# Autodesk Inventor assembly: SerenityMk2Complete
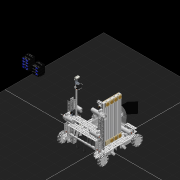
[picture p0: Inventor's stored thumbnail of the model, 180x180]
Saved by Autodesk Inventor 2015 SP1 (Build 190203100, 203)
## iProperties
Created: 2015-01-22
Part Number: SerenityMk2Complete
Document SubType Name: Assembly
Designer: rihoobler
Author: rihoobler
## Documents named in this file (41)
- C:\Users\datenney\Documents\GitHub\CAD\SerenityMk.2\SerenityMk2Complete.iam
- C:\Users\datenney\Documents\GitHub\CAD\SerenityMk.2\Frame.iam
- C:\Users\datenney\Documents\GitHub\CAD\SerenityMk.2\Normal Wheel Assembly.iam
- C:\Users\datenney\Documents\GitHub\CAD\SerenityMk.2\Omni Assembly.iam
- C:\Users\datenney\Documents\GitHub\CAD\SerenityMk.2\Imported Components\tetrix_739172_2012\tetrix_739172_2012.iam
- C:\Users\datenney\Documents\GitHub\CAD\SerenityMk.2\20X40long.ipt
- C:\Users\datenney\Documents\GitHub\CAD\SerenityMk.2\Slider.ipt
- C:\Users\datenney\Documents\GitHub\CAD\SerenityMk.2\Imported Components\tetrix_739067_2012_160_channel\tetrix_739067_2012_160_channel.ipt
- C:\Users\datenney\Documents\GitHub\CAD\SerenityMk.2\SlideAssembly.iam
- C:\Users\datenney\Documents\GitHub\CAD\SerenityMk.2\20x20extrusion.ipt
- C:\Users\datenney\Documents\GitHub\CAD\SerenityMk.2\spool.ipt
- C:\Users\datenney\Documents\GitHub\CAD\SerenityMk.2\20x20extrusionshort.ipt
- C:\Users\datenney\Documents\GitHub\CAD\SerenityMk.2\Imported Components\tetrix_739062_2012\tetrix_739062_2012.ipt
- C:\Users\datenney\Documents\GitHub\CAD\SerenityMk.2\Bucket.ipt
- C:\Users\datenney\Documents\GitHub\CAD\SerenityMk.2\Bucket Flap.ipt
- C:\Users\datenney\Documents\GitHub\CAD\SerenityMk.2\Imported Components\tetrix_739060_2012\tetrix_739060_2012.ipt
- C:\Users\datenney\Documents\GitHub\CAD\SerenityMk.2\Imported Components\tetrix_739197_2012\tetrix_739197_2012.iam
- C:\Users\datenney\Documents\GitHub\CAD\SerenityMk.2\Flat-7.ipt
- C:\Users\datenney\Documents\GitHub\CAD\SerenityMk.2\Imported Components\tetrix_739066_2012_96_channel\tetrix_739066_2012_96_channel.ipt
- C:\Users\datenney\Documents\GitHub\CAD\SerenityMk.2\ramp.ipt
- C:\Users\datenney\Documents\GitHub\CAD\SerenityMk.2\Imported Components\tetrix_739069_2012_416_channel\tetrix_739069_2012_416_channel.ipt
- C:\Users\datenney\Documents\GitHub\CAD\SerenityMk.2\Imported Components\tetrix_739068_2012_288_channel\tetrix_739068_2012_288_channel.ipt
- C:\Users\datenney\Documents\GitHub\CAD\SerenityMk.2\Imported Components\tetrix_739091_2012\tetrix_739091_2012.ipt
- C:\Users\datenney\Documents\GitHub\CAD\SerenityMk.2\sweeper.iam
- C:\Users\datenney\Documents\GitHub\CAD\SerenityMk.2\Imported Components\tetrix_739070_2012\tetrix_739070_2012.ipt
- C:\Users\datenney\Documents\GitHub\CAD\SerenityMk.2\Imported Components\sensor_light_2012\sensor_light_2012.ipt
- C:\Users\datenney\Documents\GitHub\CAD\SerenityMk.2\Imported Components\tetrix_739072_2012\tetrix_739072_2012.ipt
- C:\Users\datenney\Documents\GitHub\CAD\SerenityMk.2\Imported Components\tetrix_739089_2012\tetrix_739089_2012.ipt
- C:\Users\datenney\Documents\GitHub\CAD\SerenityMk.2\LiftSpool.ipt
- C:\Users\datenney\Documents\GitHub\CAD\COTSParts\Tetrix\Tetrix DC motor controller.ipt
- C:\Users\datenney\Documents\GitHub\CAD\COTSParts\Tetrix\NXT brick.ipt
- C:\Users\datenney\Documents\GitHub\CAD\COTSParts\Tetrix\NXT battery cover.ipt
- C:\Users\datenney\Documents\GitHub\CAD\COTSParts\Tetrix\Tetrix servo controller.ipt
- C:\Users\datenney\Documents\GitHub\CAD\COTSParts\Tetrix\Tetrix power switch.ipt
- C:\Users\datenney\Documents\GitHub\CAD\SerenityMk.2\Tetrix flat bar 257.175 mm.ipt
- C:\Users\datenney\Documents\GitHub\CAD\SerenityMk.2\Imported Components\tetrix_739197_2012\TETRIX_739197_SERVO_2012.ipt
- C:\Users\datenney\Documents\GitHub\CAD\SerenityMk.2\Imported Components\tetrix_739197_2012\TETRIX_739197_METAL_HORN_2012.ipt
- C:\Users\datenney\Documents\GitHub\CAD\SerenityMk.2\Imported Components\tetrix_739197_2012\TETRIX_739197_SCREW_2012.ipt
- C:\Users\datenney\Documents\GitHub\CAD\SerenityMk.2\Imported Components\tetrix_739197_2012\TETRIX_739197_PLASTIC_HORN_2012.ipt
- C:\Users\datenney\Documents\GitHub\CAD\SerenityMk.2\The Law Head.ipt
- C:\Users\datenney\Documents\GitHub\CAD\Imported Components\am-2964NeveRest\am-2964NeveRest.ipt
## Components (99 placed, 40 different names)
1. Frame:1 [sub-assembly] — Insert:1, Insert:2, Insert:3, Insert:4, Insert:5, Insert:6, Insert:7, Insert:8, Insert:9, Insert:10, Insert:11, Insert:12, Insert:13, Insert:14, Insert:15, Insert:16, Mate:1, Mate:2, Flush:1, Mate:6, Flush:5, Mate:7, Mate:33, Mate:34, Mate:35, Mate:42, Mate:43, Angle:8, Mate:44, Mate:45, Flush:26, Flush:27, Mate:55, Flush:29, Mate:75, Mate:76, Angle:15, Mate:84, Mate:85, Mate:86, Mate:94, Mate:95, Angle:18, Mate:111
2. Normal Wheel Assembly:1 [sub-assembly] — Insert:1
3. Normal Wheel Assembly:2 [sub-assembly] — Insert:2
4. Normal Wheel Assembly:3 [sub-assembly] — Insert:4
5. Normal Wheel Assembly:4 [sub-assembly] — Insert:3
6. Omni Assembly:1 [sub-assembly] — Insert:6, Mate:107
7. Omni Assembly:2 [sub-assembly] — Insert:5, Mate:108
8. Omni Assembly:3 [sub-assembly] — Insert:8, Mate:107, Rotation:1
9. Omni Assembly:4 [sub-assembly] — Insert:7, Mate:108, Rotation:1
10. tetrix_739172_2012:1 [sub-assembly] — Insert:9
11. tetrix_739172_2012:2 [sub-assembly] — Insert:10
12. tetrix_739172_2012:3 [sub-assembly] — Insert:11
13. tetrix_739172_2012:4 [sub-assembly] — Insert:12
14. tetrix_739172_2012:5 [sub-assembly] — Insert:15
15. tetrix_739172_2012:6 [sub-assembly] — Insert:16
16. tetrix_739172_2012:7 [sub-assembly] — Insert:13
17. tetrix_739172_2012:8 [sub-assembly] — Insert:14
18. 20X40long:1 — Mate:1, Mate:2, Flush:1, Flush:2, Mate:3, Mate:4, Mate:5, Mate:8, Mate:96, Mate:97, Flush:38
19. Slider:1 — Flush:2, Mate:3, Mate:4, Flush:4, Angle:1, Mate:9, Flush:7, Insert:17, Flush:44
20. Slider:2 — Flush:4, Mate:5, Flush:44
21. tetrix_739067_2012_160_channel:1 — Mate:6, Flush:5, Mate:7, Mate:74, Flush:28
22. SlideAssembly:1 [sub-assembly] — Angle:1, Mate:8, Mate:9, Flush:7, Angle:2, Mate:10, Flush:8, Mate:11, Insert:18
23. SlideAssembly:2 [sub-assembly] — Angle:2, Mate:10, Flush:8, Mate:11, Angle:3, Flush:9, Flush:10, Mate:12, Insert:19, Insert:20
24. SlideAssembly:3 [sub-assembly] — Angle:3, Flush:9, Flush:10, Mate:12, Angle:4, Flush:14, Flush:15, Mate:17, Insert:21, Insert:22
25. 20x20extrusion:1 — Mate:13, Mate:14, Flush:11, Mate:15, Mate:16, Flush:16, Mate:18, Flush:18
26. Slider:3 — Mate:13, Mate:14, Flush:11, Flush:12, Flush:13, Flush:14, Flush:15, Mate:17, Insert:23
27. Slider:4 — Flush:12, Flush:13, Mate:15, Mate:16, Angle:4
28. spool:1 — Insert:18
29. spool:2 — Insert:17
30. spool:3 — Insert:19
31. spool:4 — Insert:20
32. spool:6 — Insert:21
33. spool:7 — Insert:22
34. spool:8 — Insert:23
35. 20x20extrusionshort:1 — Flush:16, Mate:18, Mate:19, Angle:5, Flush:17, Flush:18, Flush:19, Mate:24, Angle:6, Flush:21
36. tetrix_739062_2012:1 — Mate:19, Angle:5, Flush:17, Mate:20, Mate:21, Mate:22
37. Bucket:1 — Mate:20, Mate:21, Mate:22, Flush:19, Flush:20, Mate:23
38. Bucket Flap:1 — Flush:20, Mate:23, Mate:31, Mate:32
39. tetrix_739060_2012:1 — Mate:24, Angle:6, Flush:21, Mate:25, Angle:7, Mate:26
40. tetrix_739197_2012:1 [sub-assembly] — Mate:25, Angle:7, Mate:26, Mate:27, Mate:28
41. Flat-7:1 — Mate:27, Mate:28, Mate:29, Mate:30
42. Flat-7:2 — Mate:29, Mate:30, Mate:31, Mate:32
43. tetrix_739066_2012_96_channel:1 — Mate:33, Mate:34, Mate:35, Mate:36, Mate:37, Mate:38
44. tetrix_739066_2012_96_channel:2 — Mate:36, Mate:37, Mate:38, Mate:39, Flush:39, Flush:40
45. ramp:1 — Mate:39, Flush:39, Flush:40
46. tetrix_739069_2012_416_channel:1 — Mate:42, Mate:43, Angle:8, Flush:22, Angle:9, Mate:46, Mate:48, Flush:24, Mate:49, Mate:56
47. tetrix_739068_2012_288_channel:1 — Flush:22, Angle:9, Mate:44, Mate:45, Mate:47, Flush:23, Mate:50, Mate:51, Flush:25, Mate:57
48. tetrix_739068_2012_288_channel:2 — Mate:46, Mate:47, Flush:23, Mate:58, Mate:59, Mate:60
49. tetrix_739068_2012_288_channel:3 — Mate:48, Flush:24, Mate:49, Mate:52, Mate:53, Mate:87, Mate:88, Mate:89, Mate:90, Mate:91, Angle:17, Mate:110, Flush:43
50. tetrix_739068_2012_288_channel:4 — Mate:50, Mate:51, Flush:25, Mate:54, Mate:92, Mate:93
51. tetrix_739066_2012_96_channel:3 — Mate:52, Mate:53, Flush:26, Angle:10, Insert:26, Insert:27
52. tetrix_739066_2012_96_channel:4 — Mate:54, Flush:27, Mate:55, Insert:24, Insert:25
53. tetrix_739068_2012_288_channel:5 — Mate:56, Angle:10, Mate:57
54. tetrix_739091_2012:1 — Insert:24
55. tetrix_739091_2012:2 — Insert:25
56. tetrix_739091_2012:3 — Insert:26, Insert:28
57. tetrix_739091_2012:4 — Insert:27
58. sweeper:1 [sub-assembly] — Insert:28
59. tetrix_739060_2012:2 — Mate:58, Mate:59, Mate:60, Mate:61, Angle:11, Mate:62
60. tetrix_739197_2012:2 [sub-assembly] — Mate:61, Angle:11, Mate:62, Mate:63, Mate:124, Mate:125
61. tetrix_739070_2012:1 — Mate:63, Mate:65, Mate:66, Mate:67, Mate:124, Mate:125
62. tetrix_739060_2012:3 — Mate:65, Mate:66, Mate:67, Mate:131, Flush:45, Mate:132
63. tetrix_739197_2012:3 [sub-assembly] — Mate:71, Mate:126, Mate:127, Mate:128, Mate:131, Flush:45, Mate:132
64. tetrix_739062_2012:2 — Mate:71, Mate:72, Mate:73, Angle:14, Mate:126, Mate:127, Mate:128
65. sensor_light_2012:1 — Mate:72, Mate:73, Angle:14
66. 20x20extrusion:2 — Mate:74, Flush:28, Flush:29
67. tetrix_739060_2012:4 — Mate:75, Mate:76, Angle:15, Mate:77, Angle:16, Mate:78
68. tetrix_739197_2012:4 [sub-assembly] — Mate:77, Angle:16, Mate:78, Mate:79, Mate:80, Mate:136, Mate:137
69. tetrix_739062_2012:3 — Mate:79, Mate:80, Mate:82, Mate:105, Mate:106, Mate:136, Mate:137
70. tetrix_739072_2012:1 — Mate:82, Mate:105, Mate:106
71. tetrix_739089_2012:1 — Mate:90, Mate:91, Angle:17, Flush:31, Mate:148, Mate:149
72. tetrix_739089_2012:2 — Flush:30, Mate:92, Mate:93, Mate:138, Mate:139
73. tetrix_739089_2012:3 — Mate:87, Mate:88, Mate:89, Flush:30, Mate:146, Mate:150
74. tetrix_739089_2012:4 — Mate:84, Mate:85, Mate:86, Mate:144, Mate:145
75. tetrix_739089_2012:5 — Mate:94, Mate:95, Angle:18, Mate:142, Mate:143
76. tetrix_739089_2012:6 — Mate:96, Mate:97, Flush:31, Mate:140, Mate:141
77. am-2964NeveRest:1 — Mate:138, Mate:139
78. am-2964NeveRest:2 — Mate:142, Mate:143
79. am-2964NeveRest:3 — Mate:146, Mate:150
80. am-2964NeveRest:4 — Mate:140, Mate:141
81. am-2964NeveRest:5 — Mate:144, Mate:145
82. am-2964NeveRest:6 — Mate:148, Mate:149
83. LiftSpool:1 — Flush:38
84. Tetrix DC motor controller:1
85. Tetrix DC motor controller:2
86. Tetrix DC motor controller:3
87. Tetrix DC motor controller:4
88. NXT brick:1 — Mate:109, Flush:41, Flush:42, Flush:43, Mate:111
89. NXT battery cover:1 — Mate:109, Flush:41, Flush:42, Mate:110
90. Tetrix servo controller:1
91. Tetrix servo controller:2
92. Tetrix servo controller:3
93. Tetrix power switch:1
94. Tetrix flat bar 257.175 mm:1 — Mate:121, Mate:122, Mate:123, Mate:133, Mate:134, Mate:135
95. TETRIX_739197_SERVO_2012:1 — Insert:29, Mate:118, Mate:120
96. TETRIX_739197_METAL_HORN_2012:1 — Mate:115, Mate:116, Mate:117, Mate:119, Mate:121, Mate:122, Mate:123, Rotation:2
97. TETRIX_739197_SCREW_2012:1 — Mate:117, Insert:29, Mate:118, Mate:119
98. TETRIX_739197_PLASTIC_HORN_2012:1 — Mate:115, Mate:116, Mate:120, Rotation:2
99. The Law Head:1 — Mate:133, Mate:134, Mate:135
## Relationships (213: Mate 129, Flush 37, Insert 29, Angle 16, RelateRotation 2)
- Insert:1: Frame:1 ↔ Normal Wheel Assembly:1
- Insert:2: Frame:1 ↔ Normal Wheel Assembly:2
- Insert:3: Frame:1 ↔ Normal Wheel Assembly:4
- Insert:4: Frame:1 ↔ Normal Wheel Assembly:3
- Insert:5: Frame:1 ↔ Omni Assembly:2
- Insert:6: Frame:1 ↔ Omni Assembly:1
- Insert:7: Frame:1 ↔ Omni Assembly:4
- Insert:8: Frame:1 ↔ Omni Assembly:3
- Insert:9: Frame:1 ↔ tetrix_739172_2012:1
- Insert:10: Frame:1 ↔ tetrix_739172_2012:2
- Insert:11: Frame:1 ↔ tetrix_739172_2012:3
- Insert:12: Frame:1 ↔ tetrix_739172_2012:4
- Insert:13: Frame:1 ↔ tetrix_739172_2012:7
- Insert:14: Frame:1 ↔ tetrix_739172_2012:8
- Insert:15: Frame:1 ↔ tetrix_739172_2012:5
- Insert:16: Frame:1 ↔ tetrix_739172_2012:6
- Mate:1: Frame:1 ↔ 20X40long:1
- Mate:2 (38.608 mm): Frame:1 ↔ 20X40long:1
- Flush:1: Frame:1 ↔ 20X40long:1
- Flush:2: 20X40long:1 ↔ Slider:1
- Mate:3: 20X40long:1 ↔ Slider:1
- Mate:4: 20X40long:1 ↔ Slider:1
- Flush:4: Slider:1 ↔ Slider:2
- Mate:5: 20X40long:1 ↔ Slider:2
- Mate:6: Frame:1 ↔ tetrix_739067_2012_160_channel:1
- Flush:5: Frame:1 ↔ tetrix_739067_2012_160_channel:1
- Mate:7: Frame:1 ↔ tetrix_739067_2012_160_channel:1
- Angle:1 (180 deg): Slider:1 ↔ SlideAssembly:1
- Mate:8: 20X40long:1 ↔ SlideAssembly:1
- Mate:9: Slider:1 ↔ SlideAssembly:1
- Flush:7: Slider:1 ↔ SlideAssembly:1
- Angle:2 (180 deg): SlideAssembly:1 ↔ SlideAssembly:2
- Mate:10: SlideAssembly:1 ↔ SlideAssembly:2
- Flush:8: SlideAssembly:1 ↔ SlideAssembly:2
- Mate:11: SlideAssembly:1 ↔ SlideAssembly:2
- Angle:3 (180 deg): SlideAssembly:2 ↔ SlideAssembly:3
- Flush:9: SlideAssembly:2 ↔ SlideAssembly:3
- Flush:10: SlideAssembly:2 ↔ SlideAssembly:3
- Mate:12: SlideAssembly:2 ↔ SlideAssembly:3
- Mate:13: 20x20extrusion:1 ↔ Slider:3
- Mate:14: 20x20extrusion:1 ↔ Slider:3
- Flush:11: 20x20extrusion:1 ↔ Slider:3
- Flush:12: Slider:3 ↔ Slider:4
- Flush:13: Slider:3 ↔ Slider:4
- Mate:15: 20x20extrusion:1 ↔ Slider:4
- Mate:16: 20x20extrusion:1 ↔ Slider:4
- Angle:4 (180 deg): SlideAssembly:3 ↔ Slider:4
- Flush:14: SlideAssembly:3 ↔ Slider:3
- Flush:15: SlideAssembly:3 ↔ Slider:3
- Mate:17: SlideAssembly:3 ↔ Slider:3
- Insert:17: Slider:1 ↔ spool:2
- Insert:18: SlideAssembly:1 ↔ spool:1
- Insert:19: SlideAssembly:2 ↔ spool:3
- Insert:20: SlideAssembly:2 ↔ spool:4
- Insert:21: SlideAssembly:3 ↔ spool:6
- Insert:22: SlideAssembly:3 ↔ spool:7
- Insert:23: Slider:3 ↔ spool:8
- Flush:16: 20x20extrusion:1 ↔ 20x20extrusionshort:1
- Mate:18: 20x20extrusion:1 ↔ 20x20extrusionshort:1
- Mate:19: 20x20extrusionshort:1 ↔ tetrix_739062_2012:1
- Angle:5 (180 deg): 20x20extrusionshort:1 ↔ tetrix_739062_2012:1
- Flush:17 (-3.5 mm): 20x20extrusionshort:1 ↔ tetrix_739062_2012:1
- Mate:20: tetrix_739062_2012:1 ↔ Bucket:1
- Mate:21: tetrix_739062_2012:1 ↔ Bucket:1
- Mate:22: tetrix_739062_2012:1 ↔ Bucket:1
- Flush:18 (-190.5 mm): 20x20extrusion:1 ↔ 20x20extrusionshort:1
- Flush:19 (-76.2 mm): 20x20extrusionshort:1 ↔ Bucket:1
- Flush:20: Bucket:1 ↔ Bucket Flap:1
- Mate:23: Bucket:1 ↔ Bucket Flap:1
- Mate:24: 20x20extrusionshort:1 ↔ tetrix_739060_2012:1
- Angle:6 (0 deg): 20x20extrusionshort:1 ↔ tetrix_739060_2012:1
- Flush:21: 20x20extrusionshort:1 ↔ tetrix_739060_2012:1
- Mate:25: tetrix_739060_2012:1 ↔ tetrix_739197_2012:1
- Angle:7 (0 deg): tetrix_739060_2012:1 ↔ tetrix_739197_2012:1
- Mate:26: tetrix_739060_2012:1 ↔ tetrix_739197_2012:1
- Mate:27: tetrix_739197_2012:1 ↔ Flat-7:1
- Mate:28: tetrix_739197_2012:1 ↔ Flat-7:1
- Mate:29: Flat-7:1 ↔ Flat-7:2
- Mate:30: Flat-7:1 ↔ Flat-7:2
- Mate:31: Bucket Flap:1 ↔ Flat-7:2
- Mate:32: Bucket Flap:1 ↔ Flat-7:2
- Mate:33: Frame:1 ↔ tetrix_739066_2012_96_channel:1
- Mate:34: Frame:1 ↔ tetrix_739066_2012_96_channel:1
- Mate:35: Frame:1 ↔ tetrix_739066_2012_96_channel:1
- Mate:36: tetrix_739066_2012_96_channel:1 ↔ tetrix_739066_2012_96_channel:2
- Mate:37: tetrix_739066_2012_96_channel:1 ↔ tetrix_739066_2012_96_channel:2
- Mate:38: tetrix_739066_2012_96_channel:1 ↔ tetrix_739066_2012_96_channel:2
- Mate:39: tetrix_739066_2012_96_channel:2 ↔ ramp:1
- Mate:42: Frame:1 ↔ tetrix_739069_2012_416_channel:1
- Mate:43: Frame:1 ↔ tetrix_739069_2012_416_channel:1
- Angle:8 (0 deg): Frame:1 ↔ tetrix_739069_2012_416_channel:1
- Flush:22: tetrix_739069_2012_416_channel:1 ↔ tetrix_739068_2012_288_channel:1
- Angle:9 (0 deg): tetrix_739069_2012_416_channel:1 ↔ tetrix_739068_2012_288_channel:1
- Mate:44: Frame:1 ↔ tetrix_739068_2012_288_channel:1
- Mate:45: Frame:1 ↔ tetrix_739068_2012_288_channel:1
- Mate:46: tetrix_739069_2012_416_channel:1 ↔ tetrix_739068_2012_288_channel:2
- Mate:47: tetrix_739068_2012_288_channel:1 ↔ tetrix_739068_2012_288_channel:2
- Flush:23: tetrix_739068_2012_288_channel:1 ↔ tetrix_739068_2012_288_channel:2
- Mate:48: tetrix_739069_2012_416_channel:1 ↔ tetrix_739068_2012_288_channel:3
- Flush:24: tetrix_739069_2012_416_channel:1 ↔ tetrix_739068_2012_288_channel:3
- Mate:49: tetrix_739069_2012_416_channel:1 ↔ tetrix_739068_2012_288_channel:3
- Mate:50: tetrix_739068_2012_288_channel:1 ↔ tetrix_739068_2012_288_channel:4
- Mate:51: tetrix_739068_2012_288_channel:1 ↔ tetrix_739068_2012_288_channel:4
- Flush:25: tetrix_739068_2012_288_channel:1 ↔ tetrix_739068_2012_288_channel:4
- Mate:52: tetrix_739068_2012_288_channel:3 ↔ tetrix_739066_2012_96_channel:3
- Mate:53: tetrix_739068_2012_288_channel:3 ↔ tetrix_739066_2012_96_channel:3
- Flush:26: Frame:1 ↔ tetrix_739066_2012_96_channel:3
- Mate:54: tetrix_739068_2012_288_channel:4 ↔ tetrix_739066_2012_96_channel:4
- Flush:27: Frame:1 ↔ tetrix_739066_2012_96_channel:4
- Mate:55: Frame:1 ↔ tetrix_739066_2012_96_channel:4
- Mate:56: tetrix_739069_2012_416_channel:1 ↔ tetrix_739068_2012_288_channel:5
- Angle:10 (0 deg): tetrix_739066_2012_96_channel:3 ↔ tetrix_739068_2012_288_channel:5
- Mate:57: tetrix_739068_2012_288_channel:1 ↔ tetrix_739068_2012_288_channel:5
- Insert:24: tetrix_739066_2012_96_channel:4 ↔ tetrix_739091_2012:1
- Insert:25: tetrix_739066_2012_96_channel:4 ↔ tetrix_739091_2012:2
- Insert:26: tetrix_739066_2012_96_channel:3 ↔ tetrix_739091_2012:3
- Insert:27: tetrix_739066_2012_96_channel:3 ↔ tetrix_739091_2012:4
- Insert:28: tetrix_739091_2012:3 ↔ sweeper:1
- Mate:58: tetrix_739068_2012_288_channel:2 ↔ tetrix_739060_2012:2
- Mate:59: tetrix_739068_2012_288_channel:2 ↔ tetrix_739060_2012:2
- Mate:60: tetrix_739068_2012_288_channel:2 ↔ tetrix_739060_2012:2
- Mate:61: tetrix_739060_2012:2 ↔ tetrix_739197_2012:2
- Angle:11 (0 deg): tetrix_739060_2012:2 ↔ tetrix_739197_2012:2
- Mate:62: tetrix_739060_2012:2 ↔ tetrix_739197_2012:2
- Mate:63: tetrix_739197_2012:2 ↔ tetrix_739070_2012:1
- Mate:65: tetrix_739070_2012:1 ↔ tetrix_739060_2012:3
- Mate:66: tetrix_739070_2012:1 ↔ tetrix_739060_2012:3
- Mate:67: tetrix_739070_2012:1 ↔ tetrix_739060_2012:3
- Mate:71: tetrix_739197_2012:3 ↔ tetrix_739062_2012:2
- Mate:72: tetrix_739062_2012:2 ↔ sensor_light_2012:1
- Mate:73: tetrix_739062_2012:2 ↔ sensor_light_2012:1
- Angle:14 (0 deg): tetrix_739062_2012:2 ↔ sensor_light_2012:1
- Mate:74: tetrix_739067_2012_160_channel:1 ↔ 20x20extrusion:2
- Flush:28 (25.4 mm): tetrix_739067_2012_160_channel:1 ↔ 20x20extrusion:2
- Flush:29 (-14.478 mm): Frame:1 ↔ 20x20extrusion:2
- Mate:75: Frame:1 ↔ tetrix_739060_2012:4
- Mate:76: Frame:1 ↔ tetrix_739060_2012:4
- Angle:15 (0 deg): Frame:1 ↔ tetrix_739060_2012:4
- Mate:77: tetrix_739060_2012:4 ↔ tetrix_739197_2012:4
- Angle:16 (0 deg): tetrix_739060_2012:4 ↔ tetrix_739197_2012:4
- Mate:78: tetrix_739060_2012:4 ↔ tetrix_739197_2012:4
- Mate:79: tetrix_739197_2012:4 ↔ tetrix_739062_2012:3
- Mate:80: tetrix_739197_2012:4 ↔ tetrix_739062_2012:3
- Mate:82: tetrix_739062_2012:3 ↔ tetrix_739072_2012:1
- Mate:84: Frame:1 ↔ tetrix_739089_2012:4
- Mate:85: Frame:1 ↔ tetrix_739089_2012:4
- Mate:86: Frame:1 ↔ tetrix_739089_2012:4
- Mate:87: tetrix_739068_2012_288_channel:3 ↔ tetrix_739089_2012:3
- Mate:88: tetrix_739068_2012_288_channel:3 ↔ tetrix_739089_2012:3
- Mate:89: tetrix_739068_2012_288_channel:3 ↔ tetrix_739089_2012:3
- Mate:90: tetrix_739068_2012_288_channel:3 ↔ tetrix_739089_2012:1
- Mate:91: tetrix_739068_2012_288_channel:3 ↔ tetrix_739089_2012:1
- Angle:17 (0 deg): tetrix_739068_2012_288_channel:3 ↔ tetrix_739089_2012:1
- Flush:30: tetrix_739089_2012:2 ↔ tetrix_739089_2012:3
- Mate:92: tetrix_739068_2012_288_channel:4 ↔ tetrix_739089_2012:2
- Mate:93: tetrix_739068_2012_288_channel:4 ↔ tetrix_739089_2012:2
- Mate:94: Frame:1 ↔ tetrix_739089_2012:5
- Mate:95: Frame:1 ↔ tetrix_739089_2012:5
- Angle:18 (0 deg): Frame:1 ↔ tetrix_739089_2012:5
- Mate:96: 20X40long:1 ↔ tetrix_739089_2012:6
- Mate:97: 20X40long:1 ↔ tetrix_739089_2012:6
- Flush:31 (-50.8 mm): tetrix_739089_2012:1 ↔ tetrix_739089_2012:6
- Flush:38 (39.37 mm): 20X40long:1 ↔ LiftSpool:1
- Mate:105: tetrix_739062_2012:3 ↔ tetrix_739072_2012:1
- Mate:106: tetrix_739062_2012:3 ↔ tetrix_739072_2012:1
- Mate:107: Omni Assembly:1 ↔ Omni Assembly:3
- Mate:108: Omni Assembly:2 ↔ Omni Assembly:4
- Rotation:1 [RelateRotation] (1 ul): Omni Assembly:3 ↔ Omni Assembly:4
- Flush:39 (-3.048 mm): tetrix_739066_2012_96_channel:2 ↔ ramp:1
- Flush:40 (15.494 mm): tetrix_739066_2012_96_channel:2 ↔ ramp:1
- Mate:109: NXT brick:1 ↔ NXT battery cover:1
- Flush:41: NXT brick:1 ↔ NXT battery cover:1
- Flush:42: NXT brick:1 ↔ NXT battery cover:1
- Mate:110: tetrix_739068_2012_288_channel:3 ↔ NXT battery cover:1
- Flush:43: tetrix_739068_2012_288_channel:3 ↔ NXT brick:1
- Mate:111 (38.1 mm): Frame:1 ↔ NXT brick:1
- Mate:115: TETRIX_739197_METAL_HORN_2012:1 ↔ TETRIX_739197_PLASTIC_HORN_2012:1
- Mate:116: TETRIX_739197_METAL_HORN_2012:1 ↔ TETRIX_739197_PLASTIC_HORN_2012:1
- Mate:117: TETRIX_739197_METAL_HORN_2012:1 ↔ TETRIX_739197_SCREW_2012:1
- Insert:29: TETRIX_739197_SERVO_2012:1 ↔ TETRIX_739197_SCREW_2012:1
- Mate:118: TETRIX_739197_SERVO_2012:1 ↔ TETRIX_739197_SCREW_2012:1
- Mate:119: TETRIX_739197_METAL_HORN_2012:1 ↔ TETRIX_739197_SCREW_2012:1
- Mate:120: TETRIX_739197_SERVO_2012:1 ↔ TETRIX_739197_PLASTIC_HORN_2012:1
- Mate:121: Tetrix flat bar 257.175 mm:1 ↔ TETRIX_739197_METAL_HORN_2012:1
- Mate:122: Tetrix flat bar 257.175 mm:1 ↔ TETRIX_739197_METAL_HORN_2012:1
- Mate:123: Tetrix flat bar 257.175 mm:1 ↔ TETRIX_739197_METAL_HORN_2012:1
- Rotation:2 [RelateRotation] (1.091 ul): TETRIX_739197_METAL_HORN_2012:1 ↔ TETRIX_739197_PLASTIC_HORN_2012:1
- Mate:124: tetrix_739197_2012:2 ↔ tetrix_739070_2012:1
- Mate:125: tetrix_739197_2012:2 ↔ tetrix_739070_2012:1
- Flush:44: Slider:1 ↔ Slider:2
- Mate:126: tetrix_739197_2012:3 ↔ tetrix_739062_2012:2
- Mate:127: tetrix_739197_2012:3 ↔ tetrix_739062_2012:2
- Mate:128: tetrix_739197_2012:3 ↔ tetrix_739062_2012:2
- Mate:131: tetrix_739060_2012:3 ↔ tetrix_739197_2012:3
- Flush:45: tetrix_739060_2012:3 ↔ tetrix_739197_2012:3
- Mate:132: tetrix_739060_2012:3 ↔ tetrix_739197_2012:3
- Mate:133: Tetrix flat bar 257.175 mm:1 ↔ The Law Head:1
- Mate:134: Tetrix flat bar 257.175 mm:1 ↔ The Law Head:1
- Mate:135: Tetrix flat bar 257.175 mm:1 ↔ The Law Head:1
- Mate:136: tetrix_739197_2012:4 ↔ tetrix_739062_2012:3
- Mate:137: tetrix_739197_2012:4 ↔ tetrix_739062_2012:3
- Mate:138: tetrix_739089_2012:2 ↔ am-2964NeveRest:1
- Mate:139: tetrix_739089_2012:2 ↔ am-2964NeveRest:1
- Mate:140: tetrix_739089_2012:6 ↔ am-2964NeveRest:4
- Mate:141: tetrix_739089_2012:6 ↔ am-2964NeveRest:4
- Mate:142: tetrix_739089_2012:5 ↔ am-2964NeveRest:2
- Mate:143: tetrix_739089_2012:5 ↔ am-2964NeveRest:2
- Mate:144: tetrix_739089_2012:4 ↔ am-2964NeveRest:5
- Mate:145: tetrix_739089_2012:4 ↔ am-2964NeveRest:5
- Mate:146: tetrix_739089_2012:3 ↔ am-2964NeveRest:3
- Mate:148: tetrix_739089_2012:1 ↔ am-2964NeveRest:6
- Mate:149: tetrix_739089_2012:1 ↔ am-2964NeveRest:6
- Mate:150: tetrix_739089_2012:3 ↔ am-2964NeveRest:3
